# Autodesk Inventor assembly: Assembly2
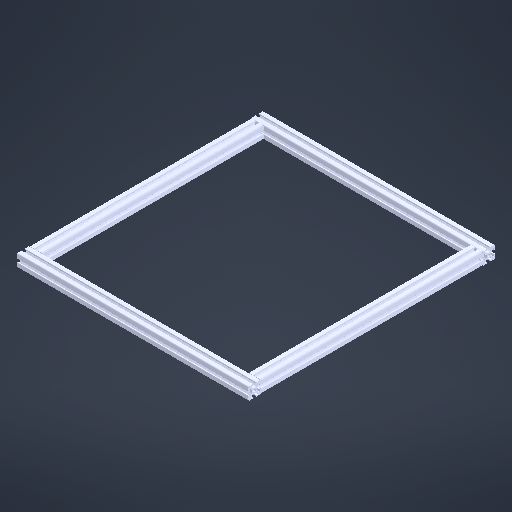
[picture p0: Inventor's stored thumbnail of the model, 512x512]
Saved by Autodesk Inventor 2026.2 (Build 302298010, 298A)
## iProperties
Created: 2026-08-09
Part Number: Assembly2
Document SubType Name: Assembly
Designer: aiden
Author: aiden
## Documents named in this file (3)
- D:\University Documents\Research - Downey\NMR and Water Qual Sys\New NMR Frame 8_7_2026\Frame\Assembly2.iam
- D:\University Documents\Research - Downey\NMR and Water Qual Sys\Water Quality Master\flowthrough-water-quality-monitoring-system-main\system_development\Moultrie\v0.3.1\CAD\NMRtray20v2\Al Bars\AL353.7_5537T104.ipt
- D:\University Documents\Research - Downey\NMR and Water Qual Sys\Water Quality Master\flowthrough-water-quality-monitoring-system-main\system_development\Moultrie\v0.3.1\CAD\NMRtray20v2\Al Bars\AL369.575_5537T104.ipt
## Components (4 placed, 2 different names)
1. AL353.7_5537T104:1 — Rigid:1, Rigid:3
2. AL369.575_5537T104:1 — Rigid:1, Rigid:2
3. AL353.7_5537T104:2 — Rigid:2
4. AL369.575_5537T104:2 — Rigid:3
## Relationships (3: WeldJoint 3)
- Rigid:1 [WeldJoint]: AL353.7_5537T104:1 ↔ AL369.575_5537T104:1
- Rigid:2 [WeldJoint]: AL369.575_5537T104:1 ↔ AL353.7_5537T104:2
- Rigid:3 [WeldJoint]: AL353.7_5537T104:1 ↔ AL369.575_5537T104:2
